# Autodesk Inventor assembly: Oring-probe-flange-with-GV
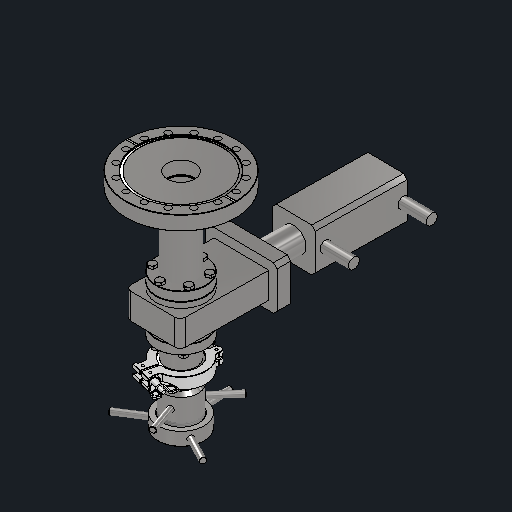
[picture p0: Inventor's stored thumbnail of the model, 512x512]
Saved by Autodesk Inventor 2027.1 (Build 311270010, 270A)
## iProperties
Created: 2024-05-30
Part Number: Oring-probe-flange-with-GV
Document SubType Name: Assembly
Designer: kuzmin
Author: kuzmin
## Documents named in this file (7)
- C:\Users\queezz\Dropbox\Drawings\pihti-cad\Plasma Vessel\Oring-probe-flange-with-GV.iam
- C:\Users\queezz\Dropbox\Drawings\pihti-cad\ContentCenter\CF-parts\CF-Flanges\CF_152-70.ipt
- C:\Users\queezz\Dropbox\Drawings\pihti-cad\ContentCenter\CF-parts\CF70-nipple\CF70-nipple.iam
- C:\Users\queezz\Dropbox\Drawings\pihti-cad\ContentCenter\CF-parts\CF70-gate-valve\Gatevalve_70_pneumatic.iam
- C:\Users\queezz\Dropbox\Drawings\pihti-cad\ContentCenter\NW\NW40_viton_centering_ring.ipt
- C:\Users\queezz\Dropbox\Drawings\pihti-cad\ContentCenter\Fastners\M6x20-HexCS.ipt
- C:\Users\queezz\Dropbox\Drawings\pihti-cad\Plasma Vessel\pipe-o-ring-gauge-port-assembly.iam
## Components (23 placed, 6 different names)
1. CF_152-70:1 — Rotational:3, Mate:2
2. CF70-nipple:1 [sub-assembly] — Rotational:3, Mate:2, Rigid:4, Rigid:5, Rigid:6, Rigid:7, Rigid:8, Rigid:9, Rigid:10, Rigid:11, Rigid:12, Rigid:13, Rigid:14, Rotational:4
3. Gatevalve_70_pneumatic:1 [sub-assembly]
4. NW40_viton_centering_ring:1
5. pipe-o-ring-gauge-port-assembly:1 [sub-assembly]
6. DIN EN 24017 M6 x 20:1 — Rigid:4
7. DIN EN 24017 M6 x 20:2 — Rigid:5
8. DIN EN 24017 M6 x 20:3 — Rigid:6
9. DIN EN 24017 M6 x 20:4 — Rigid:8
10. DIN EN 24017 M6 x 20:5 — Rigid:9
11. DIN EN 24017 M6 x 20:6 — Rigid:7
12. DIN EN 24017 M6 x 20:7
13. DIN EN 24017 M6 x 20:8 — Rigid:12
14. DIN EN 24017 M6 x 20:9 — Rigid:11
15. DIN EN 24017 M6 x 20:10 — Rigid:10
16. DIN EN 24017 M6 x 20:11 — Rigid:13
17. DIN EN 24017 M6 x 20:12 — Rigid:14
18. DIN EN 24017 M6 x 20:13
19. DIN EN 24017 M6 x 20:14
20. DIN EN 24017 M6 x 20:15
21. DIN EN 24017 M6 x 20:16
22. DIN EN 24017 M6 x 20:17 — Rotational:4
23. DIN EN 24017 M6 x 20:18
## Relationships (26: WeldJoint 18, RevoluteJoint 5, Mate 2, Flush 1)
- Rotational:3 [RevoluteJoint]: CF_152-70:1 ↔ CF70-nipple:1
- [RevoluteJoint]: CF70-nipple:1 ↔ Gatevalve_70_pneumatic:1
- [RevoluteJoint]: Gatevalve_70_pneumatic:1 ↔ pipe-o-ring-gauge-port-assembly:1
- [WeldJoint]: NW40_viton_centering_ring:1 ↔ pipe-o-ring-gauge-port-assembly:1
- [WeldJoint]: NW40_viton_centering_ring:1 ↔ pipe-o-ring-gauge-port-assembly:1
- [Mate]: NW40_viton_centering_ring:1 ↔ pipe-o-ring-gauge-port-assembly:1
- [Flush]: NW40_viton_centering_ring:1 ↔ pipe-o-ring-gauge-port-assembly:1
- Mate:2: CF_152-70:1 ↔ CF70-nipple:1
- Rigid:4 [WeldJoint]: CF70-nipple:1 ↔ DIN EN 24017 M6 x 20:1
- Rigid:5 [WeldJoint]: CF70-nipple:1 ↔ DIN EN 24017 M6 x 20:2
- Rigid:6 [WeldJoint]: CF70-nipple:1 ↔ DIN EN 24017 M6 x 20:3
- Rigid:7 [WeldJoint]: CF70-nipple:1 ↔ DIN EN 24017 M6 x 20:6
- Rigid:8 [WeldJoint]: CF70-nipple:1 ↔ DIN EN 24017 M6 x 20:4
- Rigid:9 [WeldJoint]: CF70-nipple:1 ↔ DIN EN 24017 M6 x 20:5
- Rigid:10 [WeldJoint]: CF70-nipple:1 ↔ DIN EN 24017 M6 x 20:10
- Rigid:11 [WeldJoint]: CF70-nipple:1 ↔ DIN EN 24017 M6 x 20:9
- Rigid:12 [WeldJoint]: CF70-nipple:1 ↔ DIN EN 24017 M6 x 20:8
- Rigid:13 [WeldJoint]: CF70-nipple:1 ↔ DIN EN 24017 M6 x 20:11
- Rigid:14 [WeldJoint]: CF70-nipple:1 ↔ DIN EN 24017 M6 x 20:12
- [WeldJoint]: pipe-o-ring-gauge-port-assembly:1 ↔ DIN EN 24017 M6 x 20:15
- [WeldJoint]: pipe-o-ring-gauge-port-assembly:1 ↔ DIN EN 24017 M6 x 20:16
- [WeldJoint]: pipe-o-ring-gauge-port-assembly:1 ↔ DIN EN 24017 M6 x 20:14
- [WeldJoint]: pipe-o-ring-gauge-port-assembly:1 ↔ DIN EN 24017 M6 x 20:13
- [WeldJoint]: pipe-o-ring-gauge-port-assembly:1 ↔ DIN EN 24017 M6 x 20:18
- Rotational:4 [RevoluteJoint]: CF70-nipple:1 ↔ DIN EN 24017 M6 x 20:17
- [RevoluteJoint]: pipe-o-ring-gauge-port-assembly:1 ↔ DIN EN 24017 M6 x 20:7
